# Autodesk Inventor assembly: A90P
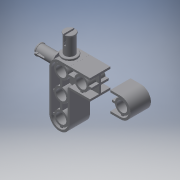
[picture p0: Inventor's stored thumbnail of the model, 180x180]
Saved by Autodesk Inventor 2019.3 (Build 233278000, 278)
## iProperties
Created: 2019-01-31
Part Number: A90P
Document SubType Name: Assembly
Designer: Varga Daniel
Vertical_hole_count: 3,000 ul
Horizontal_hole_count: 4,000 ul
Author: Varga Daniel
## Documents named in this file (7)
- C:\!_Dani\!_cloud\OneDrive\!_munka\Revolution\RevvyDemoKit\Structural parts\Connector Boxes\Connector triangle\CT2+x2+.iam
- C:\!_Dani\!_cloud\OneDrive\!_munka\Revolution\RevvyDemoKit\Structural parts\Beams\Angled Beams\Bent beam base.ipt
- C:\!_Dani\!_cloud\OneDrive\!_munka\Revolution\RevvyDemoKit\Structural parts\Beams\beam_single_end_part.ipt
- C:\!_Dani\!_cloud\OneDrive\!_munka\Revolution\RevvyDemoKit\Structural parts\Beams\beam_single_inner_part.ipt
- C:\!_Dani\!_cloud\OneDrive\!_munka\Revolution\RevvyDemoKit\Structural parts\Beams\Angled Beams\Bent beam base\Bent beam base-90.ipt
- C:\!_Dani\!_cloud\OneDrive\!_munka\Revolution\RevvyDemoKit\Structural parts\Connetor Pins\Connector_pin_collar.ipt
- C:\!_Dani\!_cloud\OneDrive\!_munka\Revolution\RevvyDemoKit\Structural parts\Connetor Pins\Connector_pin_stick.ipt
## Components (9 placed, 5 different names)
1. Bent beam base-90:1 — Flush:1, Flush:2, Flush:3, Flush:4, Mate:1, Mate:2, Flush:5, Flush:6, Mate:3, Flush:7, Flush:8, Mate:4, Mate:9, Mate:10, Flush:9, Flush:10, Mate:12, Mate:14, Angle:1, Angle:2
2. beam_single_end_part:1 — Flush:3, Flush:4, Mate:1
3. beam_single_end_part:2 — Flush:5, Flush:6, Mate:3
4. beam_single_inner_part:1 — Flush:7, Flush:8, Mate:4
5. beam_single_inner_part:2 — Flush:1, Flush:2, Mate:2
6. Connector_pin_collar:1 — Mate:5, Mate:6, Mate:10
7. Connector_pin_collar:2 — Mate:7, Mate:8, Mate:9
8. Connector_pin_stick:1 — Mate:7, Mate:8, Mate:15, Angle:2
9. Connector_pin_stick:2 — Mate:5, Mate:6, Mate:16, Angle:1
## Relationships (28: Mate 16, Flush 10, Angle 2)
- Flush:1: Bent beam base-90:1 ↔ beam_single_inner_part:2
- Flush:2: Bent beam base-90:1 ↔ beam_single_inner_part:2
- Flush:3: Bent beam base-90:1 ↔ beam_single_end_part:1
- Flush:4: Bent beam base-90:1 ↔ beam_single_end_part:1
- Mate:1 (20 mm): Bent beam base-90:1 ↔ beam_single_end_part:1
- Mate:2: Bent beam base-90:1 ↔ beam_single_inner_part:2
- Flush:5: Bent beam base-90:1 ↔ beam_single_end_part:2
- Flush:6: Bent beam base-90:1 ↔ beam_single_end_part:2
- Mate:3 (10 mm): Bent beam base-90:1 ↔ beam_single_end_part:2
- Flush:7: Bent beam base-90:1 ↔ beam_single_inner_part:1
- Flush:8: Bent beam base-90:1 ↔ beam_single_inner_part:1
- Mate:4: Bent beam base-90:1 ↔ beam_single_inner_part:1
- Mate:5: Connector_pin_collar:1 ↔ Connector_pin_stick:2
- Mate:6: Connector_pin_collar:1 ↔ Connector_pin_stick:2
- Mate:7: Connector_pin_collar:2 ↔ Connector_pin_stick:1
- Mate:8: Connector_pin_collar:2 ↔ Connector_pin_stick:1
- Mate:9: Bent beam base-90:1 ↔ Connector_pin_collar:2
- Mate:10: Bent beam base-90:1 ↔ Connector_pin_collar:1
- Flush:9 (-5 mm): Bent beam base-90:1
- Flush:10 (-5 mm): Bent beam base-90:1
- Mate:11
- Mate:12: Bent beam base-90:1
- Mate:13
- Mate:14: Bent beam base-90:1
- Mate:15: Connector_pin_stick:1
- Mate:16: Connector_pin_stick:2
- Angle:1 (0 deg): Bent beam base-90:1 ↔ Connector_pin_stick:2
- Angle:2 (0 deg): Bent beam base-90:1 ↔ Connector_pin_stick:1
